# Autodesk Inventor assembly: StrainWaveGearbox
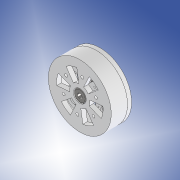
[picture p0: Inventor's stored thumbnail of the model, 180x180]
Saved by Autodesk Inventor 2017 (Build 210142000, 142)
## iProperties
Created: 2017-07-11
Part Number: StrainWaveGearbox
Document SubType Name: Assembly
Designer: zallen
Author: zallen
## Documents named in this file (8)
- C:\Users\zallen\Documents\GitHub\cr-laundry-robot\lib\Strain Wave Gearbox\StrainWaveGearbox.iam
- C:\Users\zallen\Documents\GitHub\cr-laundry-robot\lib\Strain Wave Gearbox\Flexspline.ipt
- C:\Users\zallen\Documents\GitHub\cr-laundry-robot\lib\Strain Wave Gearbox\Basespline.ipt
- C:\Users\zallen\Documents\GitHub\cr-laundry-robot\lib\Strain Wave Gearbox\WaveGenerator.ipt
- C:\Users\zallen\Documents\GitHub\cr-laundry-robot\lib\Strain Wave Gearbox\FlexsplineCover.ipt
- C:\Users\zallen\Documents\GitHub\cr-laundry-robot\lib\Strain Wave Gearbox\22x8x8mm Bearing.ipt
- C:\Users\zallen\Documents\GitHub\cr-laundry-robot\lib\Strain Wave Gearbox\WaveGeneratorRoller.ipt
- C:\Users\zallen\Documents\GitHub\cr-laundry-robot\lib\Strain Wave Gearbox\WaveGeneratorCover.ipt
## Components (11 placed, 7 different names)
1. Flexspline:1 — Mate:1, Mate:6, Mate:8, Mate:9, Mate:10
2. Basespline:1 — Mate:1, Flush:2, Mate:2, Mate:3, Mate:4, Rotation:1, Mate:6, Mate:7, Flush:3, Mate:15
3. WaveGenerator:1 — Mate:4, Rotation:1, Mate:15, Mate:16, Mate:17, Mate:18, Mate:20, Mate:21, Mate:22, Mate:23, Mate:24
4. FlexsplineCover:1 — Mate:8, Mate:9, Mate:10, Mate:11
5. 22x8x8mm Bearing:1 — Mate:7, Flush:3
6. 22x8x8mm Bearing:2 — Mate:11
7. 22x8x8mm Bearing:3 — Mate:13, Mate:16, Mate:18
8. WaveGeneratorRoller:1 — Mate:13, Mate:17
9. WaveGeneratorRoller:2 — Mate:19, Flush:4, Mate:20, Mate:21
10. 22x8x8mm Bearing:4 — Mate:19, Flush:4
11. WaveGeneratorCover:1 — Mate:22, Mate:23, Mate:24
## Relationships (25: Mate 21, Flush 3, RelateRotation 1)
- Mate:1: Flexspline:1 ↔ Basespline:1
- Flush:2: Basespline:1
- Mate:2: Basespline:1
- Mate:3: Basespline:1
- Mate:4: Basespline:1 ↔ WaveGenerator:1
- Rotation:1 [RelateRotation] (0.0217 ul): Basespline:1 ↔ WaveGenerator:1
- Mate:6: Flexspline:1 ↔ Basespline:1
- Mate:7: Basespline:1 ↔ 22x8x8mm Bearing:1
- Flush:3: Basespline:1 ↔ 22x8x8mm Bearing:1
- Mate:8: Flexspline:1 ↔ FlexsplineCover:1
- Mate:9: Flexspline:1 ↔ FlexsplineCover:1
- Mate:10: Flexspline:1 ↔ FlexsplineCover:1
- Mate:11: FlexsplineCover:1 ↔ 22x8x8mm Bearing:2
- Mate:13: 22x8x8mm Bearing:3 ↔ WaveGeneratorRoller:1
- Mate:15: Basespline:1 ↔ WaveGenerator:1
- Mate:16: WaveGenerator:1 ↔ 22x8x8mm Bearing:3
- Mate:17: WaveGenerator:1 ↔ WaveGeneratorRoller:1
- Mate:18: WaveGenerator:1 ↔ 22x8x8mm Bearing:3
- Mate:19: WaveGeneratorRoller:2 ↔ 22x8x8mm Bearing:4
- Flush:4: WaveGeneratorRoller:2 ↔ 22x8x8mm Bearing:4
- Mate:20: WaveGenerator:1 ↔ WaveGeneratorRoller:2
- Mate:21: WaveGenerator:1 ↔ WaveGeneratorRoller:2
- Mate:22: WaveGenerator:1 ↔ WaveGeneratorCover:1
- Mate:23: WaveGenerator:1 ↔ WaveGeneratorCover:1
- Mate:24: WaveGenerator:1 ↔ WaveGeneratorCover:1
